# Autodesk Inventor assembly: MSI-100
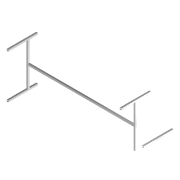
[picture p0: Inventor's stored thumbnail of the model, 180x180]
Saved by Autodesk Inventor 2020.3 (Build 243373000, 373)
## iProperties
Created: 2021-02-10
Part Number: MSI-100
Document SubType Name: Assembly
Designer: Adriano
Author: Adriano
## Documents named in this file (4)
- C:\Users\Adriano\Documents\Inventor\Mesa_Inox\MSI-100.iam
- C:\Users\Adriano\Documents\Inventor\Mesa_Inox\MSI-101.ipt
- C:\Users\Adriano\Documents\Inventor\Mesa_Inox\MSI-102.ipt
- C:\Users\Adriano\Documents\Inventor\Mesa_Inox\MSI-103.ipt
## Components (7 placed, 3 different names)
1. MSI-101:1 — Coincidência:2, Coincidência:9, Alinhamento:4
2. MSI-101:2 — Coincidência:1, Coincidência:10, Alinhamento:3
3. MSI-101:3 — Coincidência:4, Coincidência:13, Alinhamento:6
4. MSI-101:4 — Coincidência:3, Coincidência:14, Alinhamento:5
5. MSI-102:1 — Coincidência:5, Coincidência:6, Coincidência:7, Coincidência:11, Coincidência:8, Coincidência:12, Coincidência:15, Alinhamento:1, Alinhamento:2
6. MSI-103:1 — Coincidência:1, Coincidência:2, Coincidência:5, Coincidência:7, Coincidência:8, Coincidência:9, Coincidência:10, Alinhamento:3, Alinhamento:4
7. MSI-103:2 — Coincidência:3, Coincidência:4, Coincidência:6, Coincidência:11, Coincidência:12, Coincidência:13, Coincidência:14, Alinhamento:5, Alinhamento:6
## Relationships (21: Mate 15, Flush 6)
- Coincidência:1 [Mate]: MSI-101:2 ↔ MSI-103:1
- Coincidência:2 [Mate]: MSI-101:1 ↔ MSI-103:1
- Coincidência:3 [Mate]: MSI-101:4 ↔ MSI-103:2
- Coincidência:4 [Mate]: MSI-101:3 ↔ MSI-103:2
- Coincidência:5 [Mate]: MSI-102:1 ↔ MSI-103:1
- Coincidência:6 [Mate]: MSI-102:1 ↔ MSI-103:2
- Coincidência:7 [Mate]: MSI-102:1 ↔ MSI-103:1
- Coincidência:11 [Mate]: MSI-102:1 ↔ MSI-103:2
- Coincidência:8 [Mate]: MSI-102:1 ↔ MSI-103:1
- Coincidência:9 [Mate]: MSI-101:1 ↔ MSI-103:1
- Coincidência:10 [Mate]: MSI-101:2 ↔ MSI-103:1
- Coincidência:12 [Mate]: MSI-102:1 ↔ MSI-103:2
- Coincidência:13 [Mate]: MSI-101:3 ↔ MSI-103:2
- Coincidência:14 [Mate]: MSI-101:4 ↔ MSI-103:2
- Coincidência:15 [Mate]: MSI-102:1
- Alinhamento:1 [Flush]: MSI-102:1
- Alinhamento:2 [Flush]: MSI-102:1
- Alinhamento:3 [Flush] (-200 mm): MSI-101:2 ↔ MSI-103:1
- Alinhamento:4 [Flush] (-200 mm): MSI-101:1 ↔ MSI-103:1
- Alinhamento:5 [Flush] (-200 mm): MSI-101:4 ↔ MSI-103:2
- Alinhamento:6 [Flush] (-200 mm): MSI-101:3 ↔ MSI-103:2
